# Autodesk Inventor assembly: OUTK_000_Assembly
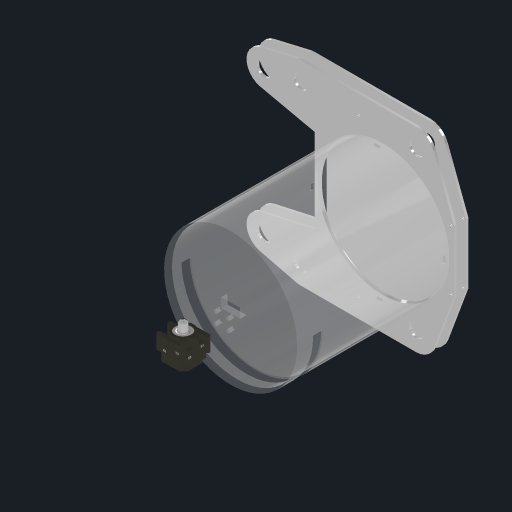
[picture p0: Inventor's stored thumbnail of the model, 512x512]
Saved by Autodesk Inventor 2024.2 (Build 282272000, 272)
## iProperties
Created: 2024-11-24
Part Number: OUTK_000_Assembly
Document SubType Name: Assembly
Designer: Bryan
Mass: 4105.44 g
Surface Area: 9606.02 cm^2
Volume: 2285.06 cm^3
Density: 1.79664 g/cm^3
Author: Bryan
## Documents named in this file (10)
- C:\Users\bobsb\OneDrive\Documents\GitHub\1622-2024-Casino-Clash-CAD-A-Thon\Outtake\OUTK_000_Assembly.iam
- C:\Users\bobsb\OneDrive\Documents\GitHub\1622-2024-Casino-Clash-CAD-A-Thon\Outtake\OUTK_002_ShotPlateNoReceptacle.ipt
- C:\Users\bobsb\OneDrive\Documents\GitHub\1622-2024-Casino-Clash-CAD-A-Thon\Outtake\OUTK_002_ShotPlateReceptacle.ipt
- C:\Users\bobsb\OneDrive\Documents\GitHub\1622-2024-Casino-Clash-CAD-A-Thon\Outtake\OUTK_001_ChipBucket.ipt
- C:\Users\bobsb\OneDrive\Documents\GitHub\1622-2024-Casino-Clash-CAD-A-Thon\Outtake\OUTK_004_PlanetaryShaft.ipt
- C:\Users\bobsb\OneDrive\Documents\GitHub\1622-2024-Casino-Clash-CAD-A-Thon\COTS Library\MAXPlanetary System\COTS_0.5inhexoutput_REV-21-2104.ipt
- C:\Users\bobsb\OneDrive\Documents\GitHub\1622-2024-Casino-Clash-CAD-A-Thon\COTS Library\MAXPlanetary System\COTS_5to1Stage_REV-21-2103.ipt
- C:\Users\bobsb\OneDrive\Documents\GitHub\1622-2024-Casino-Clash-CAD-A-Thon\COTS Library\MAXPlanetary System\COTS_InputStage_REV-21-2106.ipt
- C:\Users\bobsb\OneDrive\Documents\GitHub\1622-2024-Casino-Clash-CAD-A-Thon\COTS Library\MAXPlanetary System\COTS_NeoShaftAdapter_REV-21-2108.ipt
- C:\Users\bobsb\OneDrive\Documents\GitHub\1622-2024-Casino-Clash-CAD-A-Thon\COTS Library\Fasteners\Bolts\Button-Head\10-32\COTS_91255A265_Button Head Hex Drive Screw.ipt
## Components (9 placed, 9 different names)
1. OUTK_002_ShotPlateNoReceptacle:1 — Mate:4, Mate:5, Mate:7
2. OUTK_002_ShotPlateReceptacle:1 — Mate:3, Mate:4, Mate:5, Mate:6, Mate:7
3. OUTK_001_ChipBucket:1 — Mate:3, Mate:6, Mate:18, Mate:19
4. OUTK_004_PlanetaryShaft:1 — Mate:8, Mate:9, Mate:10
5. COTS_0.5inhexoutput_REV-21-2104:1 — Mate:8, Mate:9, Mate:11, Mate:12, Flush:1, Mate:13, Mate:18, Mate:19
6. COTS_5to1Stage_REV-21-2103:1 — Mate:12, Flush:1, Mate:13, Flush:2, Mate:14, Mate:15, Mate:16, Mate:17
7. COTS_InputStage_REV-21-2106:1 — Flush:2, Mate:14, Mate:17
8. COTS_NeoShaftAdapter_REV-21-2108:1 — Mate:15, Mate:16
9. COTS_91255A265_Button Head Hex Drive Screw:1 — Mate:10, Mate:11
## Relationships (19: Mate 17, Flush 2)
- Mate:3: OUTK_002_ShotPlateReceptacle:1 ↔ OUTK_001_ChipBucket:1
- Mate:4: OUTK_002_ShotPlateNoReceptacle:1 ↔ OUTK_002_ShotPlateReceptacle:1
- Mate:5: OUTK_002_ShotPlateNoReceptacle:1 ↔ OUTK_002_ShotPlateReceptacle:1
- Mate:6: OUTK_002_ShotPlateReceptacle:1 ↔ OUTK_001_ChipBucket:1
- Mate:7 (19.05 mm): OUTK_002_ShotPlateNoReceptacle:1 ↔ OUTK_002_ShotPlateReceptacle:1
- Mate:8: OUTK_004_PlanetaryShaft:1 ↔ COTS_0.5inhexoutput_REV-21-2104:1
- Mate:9: OUTK_004_PlanetaryShaft:1 ↔ COTS_0.5inhexoutput_REV-21-2104:1
- Mate:10: OUTK_004_PlanetaryShaft:1 ↔ COTS_91255A265_Button Head Hex Drive Screw:1
- Mate:11: COTS_0.5inhexoutput_REV-21-2104:1 ↔ COTS_91255A265_Button Head Hex Drive Screw:1
- Mate:12: COTS_0.5inhexoutput_REV-21-2104:1 ↔ COTS_5to1Stage_REV-21-2103:1
- Flush:1: COTS_0.5inhexoutput_REV-21-2104:1 ↔ COTS_5to1Stage_REV-21-2103:1
- Mate:13: COTS_0.5inhexoutput_REV-21-2104:1 ↔ COTS_5to1Stage_REV-21-2103:1
- Flush:2: COTS_5to1Stage_REV-21-2103:1 ↔ COTS_InputStage_REV-21-2106:1
- Mate:14: COTS_5to1Stage_REV-21-2103:1 ↔ COTS_InputStage_REV-21-2106:1
- Mate:15: COTS_5to1Stage_REV-21-2103:1 ↔ COTS_NeoShaftAdapter_REV-21-2108:1
- Mate:16: COTS_5to1Stage_REV-21-2103:1 ↔ COTS_NeoShaftAdapter_REV-21-2108:1
- Mate:17: COTS_5to1Stage_REV-21-2103:1 ↔ COTS_InputStage_REV-21-2106:1
- Mate:18: OUTK_001_ChipBucket:1 ↔ COTS_0.5inhexoutput_REV-21-2104:1
- Mate:19: OUTK_001_ChipBucket:1 ↔ COTS_0.5inhexoutput_REV-21-2104:1
